# Autodesk Inventor assembly: servo motor HS-7955TG
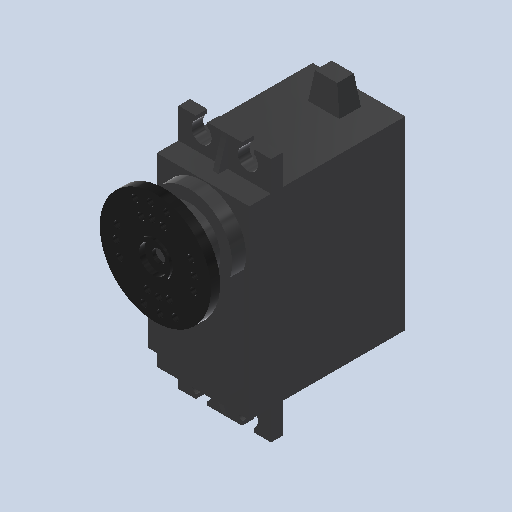
[picture p0: Inventor's stored thumbnail of the model, 512x512]
Saved by Autodesk Inventor 2022 (Build 260153000, 153)
## iProperties
Created: 2017-12-19
Part Number: servo motor HS-7955TG
Document SubType Name: Assembly
Designer: s41607
Author: s41607
## Documents named in this file (3)
- C:\Users\david\OneDrive\Documents\Singapore Polytechnic\SP-RITE\WRO FE 2024 (Repository)\models\Vehicle Model\servo motor HS-7955TG.iam
- C:\Users\david\OneDrive\Documents\Singapore Polytechnic\SP-RITE\WRO FE 2024 (Repository)\models\Vehicle Model\servo motor HS-7955TG.ipt
- C:\Users\david\OneDrive\Documents\Singapore Polytechnic\SP-RITE\WRO FE 2024 (Repository)\models\Vehicle Model\servo motor HS-7955TG round horn.ipt
## Components (2 placed, 2 different names)
1. servo motor HS-7955TG:1 — Flush:1, Flush:2, Flush:3, Insert:1
2. servo motor HS-7955TG round horn:1 — Insert:1
## Relationships (4: Flush 3, Insert 1)
- Flush:1: servo motor HS-7955TG:1
- Flush:2: servo motor HS-7955TG:1
- Flush:3: servo motor HS-7955TG:1
- Insert:1: servo motor HS-7955TG:1 ↔ servo motor HS-7955TG round horn:1
